# Autodesk Inventor assembly: Portaplanetas
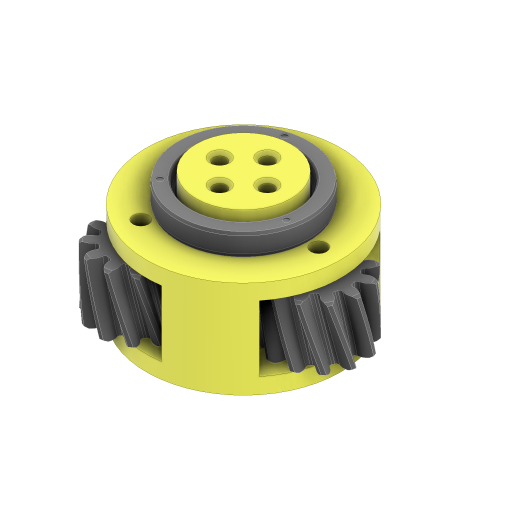
[picture p0: Inventor's stored thumbnail of the model, 512x512]
Saved by Autodesk Inventor 2024.3 (Build 283343000, 343)
## iProperties
Created: 2025-03-05
Part Number: Portaplanetas
Document SubType Name: Assembly
Designer: danie
Author: danie
## Documents named in this file (6)
- C:\Users\danie\OneDrive\Documentos\Inventor\Motor_drive\Portaplanetas.iam
- C:\Users\danie\OneDrive\Documentos\Inventor\Motor_drive\Planeta\Planeta\Planeta.ipt
- C:\Users\danie\OneDrive\Documentos\Inventor\Motor_drive\Portaplanetas2.ipt
- C:\Users\danie\OneDrive\Documentos\Inventor\Motor_drive\CR 30x42x7\CR 30x42x7\CR 30x42x7.ipt
- C:\Users\danie\OneDrive\Documentos\Inventor\Motor_drive\bearing10X15X4.ipt
- C:\Users\danie\OneDrive\Documentos\Inventor\Motor_drive\Sol\Sol\Sol.ipt
## Components (7 placed, 5 different names)
1. Planeta:1 — Mate:2, Mate:6
2. Planeta:2 — Mate:1, Mate:7
3. Planeta:3 — Mate:3, Mate:8
4. Portaplanetas2:1 — Mate:1, Mate:2, Mate:3, Mate:4, Flush:1, Mate:5, Mate:6, Mate:7, Mate:8, Mate:9, Mate:10, Mate:11, Mate:13
5. CR 30x42x7:1 — Mate:9, Mate:10
6. bearing10X15X4:1 — Mate:11, Mate:12
7. Sol:1 — Mate:12, Mate:13
## Relationships (14: Mate 13, Flush 1)
- Mate:1: Planeta:2 ↔ Portaplanetas2:1
- Mate:2: Planeta:1 ↔ Portaplanetas2:1
- Mate:3: Planeta:3 ↔ Portaplanetas2:1
- Mate:4: Portaplanetas2:1
- Flush:1: Portaplanetas2:1
- Mate:5: Portaplanetas2:1
- Mate:6: Planeta:1 ↔ Portaplanetas2:1
- Mate:7: Planeta:2 ↔ Portaplanetas2:1
- Mate:8: Planeta:3 ↔ Portaplanetas2:1
- Mate:9: Portaplanetas2:1 ↔ CR 30x42x7:1
- Mate:10: Portaplanetas2:1 ↔ CR 30x42x7:1
- Mate:11: Portaplanetas2:1 ↔ bearing10X15X4:1
- Mate:12: bearing10X15X4:1 ↔ Sol:1
- Mate:13: Portaplanetas2:1 ↔ Sol:1
